# Autodesk Inventor assembly: CNC Models
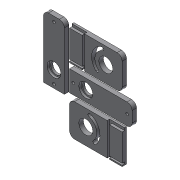
[picture p0: Inventor's stored thumbnail of the model, 180x180]
Saved by Autodesk Inventor 2018.3 (Build 223284000, 284)
## iProperties
Created: 2019-04-16
Part Number: CNC Models
Document SubType Name: Assembly
Designer: aye06091
Mass: 45.9558 g
Surface Area: 246.275 cm^2
Volume: 45.9558 cm^3
Density: 1 g/cm^3
Author: aye06091
## Documents named in this file (4)
- Y:\DeSimony-R\Senior R&D\4 R&D Shared Folder\VisiStick\VisiStick (Inventor)\Case Final - Copy\CNC Models.iam
- Y:\DeSimony-R\Senior R&D\4 R&D Shared Folder\VisiStick\VisiStick (Inventor)\Physical Parts\Lidar Sensor Case v4 Piece 2.ipt
- Y:\DeSimony-R\Senior R&D\4 R&D Shared Folder\VisiStick\VisiStick (Inventor)\Physical Parts\Lidar Sensor Case v4 Piece 1.ipt
- Y:\DeSimony-R\Senior R&D\4 R&D Shared Folder\VisiStick\VisiStick (Inventor)\Physical Parts\Lidar Sensor Case v4 Piece 3.ipt
## Components (4 placed, 3 different names)
1. Lidar Sensor Case v4 Piece 2:1 — Flush:11, Flush:16, Mate:2, Mate:3, Flush:18
2. Lidar Sensor Case v4 Piece 1:1 — Flush:17, Mate:3, Flush:18
3. Lidar Sensor Case v4 Piece 3:1 — Flush:11, Flush:14, Flush:15, Mate:1
4. Lidar Sensor Case v4 Piece 1:2 — Flush:14, Flush:15, Mate:1, Flush:16, Mate:2, Flush:17
## Relationships (9: Flush 6, Mate 3)
- Flush:11: Lidar Sensor Case v4 Piece 2:1 ↔ Lidar Sensor Case v4 Piece 3:1
- Flush:14: Lidar Sensor Case v4 Piece 3:1 ↔ Lidar Sensor Case v4 Piece 1:2
- Flush:15: Lidar Sensor Case v4 Piece 3:1 ↔ Lidar Sensor Case v4 Piece 1:2
- Mate:1 (6.604 mm): Lidar Sensor Case v4 Piece 3:1 ↔ Lidar Sensor Case v4 Piece 1:2
- Flush:16: Lidar Sensor Case v4 Piece 2:1 ↔ Lidar Sensor Case v4 Piece 1:2
- Mate:2 (6.604 mm): Lidar Sensor Case v4 Piece 2:1 ↔ Lidar Sensor Case v4 Piece 1:2
- Flush:17: Lidar Sensor Case v4 Piece 1:1 ↔ Lidar Sensor Case v4 Piece 1:2
- Mate:3 (6.604 mm): Lidar Sensor Case v4 Piece 2:1 ↔ Lidar Sensor Case v4 Piece 1:1
- Flush:18: Lidar Sensor Case v4 Piece 2:1 ↔ Lidar Sensor Case v4 Piece 1:1
